# Autodesk Inventor assembly: engine moving
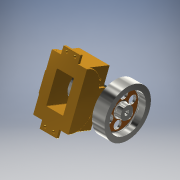
[picture p0: Inventor's stored thumbnail of the model, 180x180]
Saved by Autodesk Inventor 2017 (Build 210142000, 142)
## iProperties
Created: 2018-11-18
Part Number: engine moving
Document SubType Name: Assembly
Designer: User
Author: User
## Documents named in this file (10)
- E:\Sahil's engine\engine moving.iam
- E:\Sahil's engine\reverse gear base cast 2.ipt
- E:\Sahil's engine\reverse gear fly wheel.ipt
- E:\Sahil's engine\reverse gear crankshaft outer rod.ipt
- E:\Sahil's engine\reverse gear crankshaft counter weight 2.ipt
- E:\Sahil's engine\reverse gear crankshaft center rod.ipt
- E:\Sahil's engine\reverse gear  upper base bearing holder 1.ipt
- E:\Sahil's engine\reverse gear lower base bearing holder.ipt
- E:\Sahil's engine\reverse gear connecting rod 1.ipt
- E:\Sahil's engine\reverse gear bearing keeper.ipt
## Components (14 placed, 9 different names)
1. reverse gear fly wheel:1 — Insert:6, Mate:2, Mate:6, Rotation:2
2. reverse gear crankshaft outer rod:1 — Insert:2, Insert:6, Mate:2, Mate:3, Insert:7, Mate:6, Mate:7, Rotation:1, Rotation:2
3. reverse gear crankshaft counter weight 2:1 — Insert:2, Insert:3, Mate:7, Rotation:1
4. reverse gear crankshaft counter weight 2:2 — Insert:4, Insert:5
5. reverse gear crankshaft center rod:1 — Insert:3, Insert:4, Insert:8
6. reverse gear crankshaft outer rod:2 — Insert:5, Mate:3
7. reverse gear  upper base bearing holder 1:1 — Mate:4, Flush:1, Flush:2, Flush:3, Flush:4
8. reverse gear lower base bearing holder:1 — Mate:4, Flush:1, Flush:2, Insert:7, Mate:5
9. reverse gear base cast 2:1 — Mate:5, Flush:3, Flush:4, Mate:9, Flush:7, Flush:8
10. reverse gear  upper base bearing holder 1:2 — Mate:8, Flush:5, Flush:6, Flush:8
11. reverse gear lower base bearing holder:2 — Mate:8, Flush:5, Flush:6, Mate:9, Flush:7
12. reverse gear connecting rod 1:1 — Mate:10, Flush:9, Flush:10, Insert:8
13. reverse gear connecting rod 1:2 — Mate:10, Flush:9, Flush:10, Mate:11, Flush:11, Flush:12
14. reverse gear bearing keeper:1 — Mate:11, Flush:11, Flush:12
## Relationships (31: Flush 12, Mate 10, Insert 7, RelateRotation 2)
- Insert:2: reverse gear crankshaft outer rod:1 ↔ reverse gear crankshaft counter weight 2:1
- Insert:3 (-5 mm): reverse gear crankshaft counter weight 2:1 ↔ reverse gear crankshaft center rod:1
- Insert:4: reverse gear crankshaft counter weight 2:2 ↔ reverse gear crankshaft center rod:1
- Insert:5 (-5 mm): reverse gear crankshaft counter weight 2:2 ↔ reverse gear crankshaft outer rod:2
- Insert:6: reverse gear fly wheel:1 ↔ reverse gear crankshaft outer rod:1
- Mate:2: reverse gear fly wheel:1 ↔ reverse gear crankshaft outer rod:1
- Mate:3: reverse gear crankshaft outer rod:1 ↔ reverse gear crankshaft outer rod:2
- Mate:4: reverse gear  upper base bearing holder 1:1 ↔ reverse gear lower base bearing holder:1
- Flush:1: reverse gear  upper base bearing holder 1:1 ↔ reverse gear lower base bearing holder:1
- Flush:2 (7 mm): reverse gear  upper base bearing holder 1:1 ↔ reverse gear lower base bearing holder:1
- Insert:7 (-15 mm): reverse gear crankshaft outer rod:1 ↔ reverse gear lower base bearing holder:1
- Mate:5: reverse gear lower base bearing holder:1 ↔ reverse gear base cast 2:1
- Flush:3 (29 mm): reverse gear  upper base bearing holder 1:1 ↔ reverse gear base cast 2:1
- Flush:4: reverse gear  upper base bearing holder 1:1 ↔ reverse gear base cast 2:1
- Mate:6: reverse gear fly wheel:1 ↔ reverse gear crankshaft outer rod:1
- Mate:7: reverse gear crankshaft outer rod:1 ↔ reverse gear crankshaft counter weight 2:1
- Rotation:1 [RelateRotation] (1 ul): reverse gear crankshaft outer rod:1 ↔ reverse gear crankshaft counter weight 2:1
- Rotation:2 [RelateRotation] (1 ul): reverse gear fly wheel:1 ↔ reverse gear crankshaft outer rod:1
- Mate:8: reverse gear  upper base bearing holder 1:2 ↔ reverse gear lower base bearing holder:2
- Flush:5 (7 mm): reverse gear  upper base bearing holder 1:2 ↔ reverse gear lower base bearing holder:2
- Flush:6: reverse gear  upper base bearing holder 1:2 ↔ reverse gear lower base bearing holder:2
- Mate:9: reverse gear base cast 2:1 ↔ reverse gear lower base bearing holder:2
- Flush:7: reverse gear base cast 2:1 ↔ reverse gear lower base bearing holder:2
- Flush:8 (29 mm): reverse gear base cast 2:1 ↔ reverse gear  upper base bearing holder 1:2
- Mate:10: reverse gear connecting rod 1:1 ↔ reverse gear connecting rod 1:2
- Flush:9: reverse gear connecting rod 1:1 ↔ reverse gear connecting rod 1:2
- Flush:10: reverse gear connecting rod 1:1 ↔ reverse gear connecting rod 1:2
- Mate:11: reverse gear connecting rod 1:2 ↔ reverse gear bearing keeper:1
- Flush:11: reverse gear connecting rod 1:2 ↔ reverse gear bearing keeper:1
- Flush:12: reverse gear connecting rod 1:2 ↔ reverse gear bearing keeper:1
- Insert:8 (5.5 mm): reverse gear crankshaft center rod:1 ↔ reverse gear connecting rod 1:1
